# Autodesk Inventor assembly: Lumbar Short
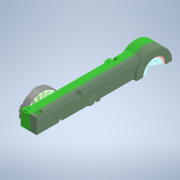
[picture p0: Inventor's stored thumbnail of the model, 180x180]
Saved by Autodesk Inventor 2022.2 (Build 262287030, 287C)
## iProperties
Created: 2022-01-12
Part Number: Lumbar Short
Document SubType Name: Assembly
Designer: Jochen
Author: Jochen
## Documents named in this file (7)
- D:\Projects\Lisbeth\CAD\Lumbar\Lumbar Short.iam
- D:\Projects\Lisbeth\CAD\Common\Motor\MotorModule.iam
- D:\Projects\Lisbeth\CAD\Common\Transmission\TransmissionPulleyCenter.iam
- D:\Projects\Lisbeth\CAD\Common\Transmission\Transmission Pulley.iam
- D:\Projects\Lisbeth\CAD\Common\Belt Tensioner\BeltTensioner 10mm.iam
- D:\Projects\Lisbeth\CAD\Common\Belt Tensioner\MotorBeltTensioner 10mm.iam
- D:\Projects\Lisbeth\CAD\Lumbar\Lumbar Short.ipt
## Components (6 placed, 6 different names)
1. MotorModule:1 [sub-assembly] — Mate:1, Mate:2, Mate:3
2. TransmissionPuileyCenter:1 [sub-assembly] — Mate:4, Mate:5
3. Transmission Pulley:1 [sub-assembly]
4. Belt tensioner:1 [sub-assembly]
5. MotorBeltTensioner:1 [sub-assembly]
6. Lumbar Short:2 — Mate:1, Mate:2, Mate:3, Mate:4, Mate:5
## Relationships (5: Mate 5)
- Mate:1: MotorModule:1 ↔ Lumbar Short:2
- Mate:2: MotorModule:1 ↔ Lumbar Short:2
- Mate:3: MotorModule:1 ↔ Lumbar Short:2
- Mate:4: TransmissionPuileyCenter:1 ↔ Lumbar Short:2
- Mate:5: TransmissionPuileyCenter:1 ↔ Lumbar Short:2
